# Autodesk Inventor assembly: B-226-2R
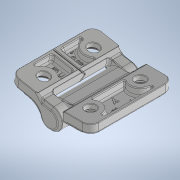
[picture p0: Inventor's stored thumbnail of the model, 180x180]
Saved by Autodesk Inventor 2021 (Build 250183000, 183)
## iProperties
Created: 2018-09-17
Part Number: B-226-2R
Document SubType Name: Assembly
Designer: brian
Sending System: PRO/ENGINEER BY PARAMETRIC TECHNOLOGY CORPORATION, 2010430
Preprocessor: PRO/ENGINEER BY PARAMETRIC TECHNOLOGY CORPORATION, 2010430
Title: CT-2136-50XXX-XX_ASM
Author: Administrator
Revision Number: 37LAST_VERSION
## Documents named in this file (4)
- C:\Users\brian\Desktop\自動主席台\新設計\阻尼鉸鏈\B-226-2R.iam
- C:\Users\brian\Desktop\自動主席台\新設計\阻尼鉸鏈\T-JL2136-50-02.ipt
- C:\Users\brian\Desktop\自動主席台\新設計\阻尼鉸鏈\T-JL2136-50-01D.ipt
- C:\Users\brian\Desktop\自動主席台\新設計\阻尼鉸鏈\T-JL2136-50-01U.ipt
## Components (3 placed, 3 different names)
1. T-JL2136-50-02_6 — 貼合:1, 貼合:2, 齊平:1, 齊平:2, 角度:1
2. T-JL2136-50-01D_7 — 貼合:1, 齊平:1, 齊平:3
3. T-JL2136-50-01U_8 — 貼合:2, 齊平:2, 齊平:3, 角度:1
## Relationships (6: Flush 3, Mate 2, Angle 1)
- 貼合:1 [Mate]: T-JL2136-50-02_6 ↔ T-JL2136-50-01D_7
- 貼合:2 [Mate]: T-JL2136-50-02_6 ↔ T-JL2136-50-01U_8
- 齊平:1 [Flush]: T-JL2136-50-02_6 ↔ T-JL2136-50-01D_7
- 齊平:2 [Flush]: T-JL2136-50-02_6 ↔ T-JL2136-50-01U_8
- 齊平:3 [Flush]: T-JL2136-50-01D_7 ↔ T-JL2136-50-01U_8
- 角度:1 [Angle] (10 deg): T-JL2136-50-02_6 ↔ T-JL2136-50-01U_8
